# Autodesk Inventor assembly: POM_T5_11
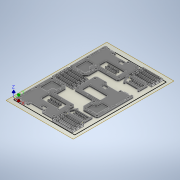
[picture p0: Inventor's stored thumbnail of the model, 180x180]
Saved by Autodesk Inventor 2022.3 (Build 263350000, 350)
## iProperties
Created: 2022-09-28
Part Number: POM_T5_11
Document SubType Name: Assembly
Designer: Masato
Author: Masato
## Documents named in this file (7)
- C:\Users\Masato\Documents\Inventor\Inventor for CIT Brains\SUSTAINA-OP\Cam\POM_T5\POM_T5_11.iam
- C:\Users\Masato\Documents\Inventor\Inventor for CIT Brains\SUSTAINA-OP\Cam\DisposableBoard.ipt
- C:\Users\Masato\Documents\Inventor\Inventor for CIT Brains\SUSTAINA-OP\UpperBody\Cockpit\Cockpit_carrier_board_frame.ipt
- C:\Users\Masato\Documents\Inventor\Inventor for CIT Brains\SUSTAINA-OP\UpperBody\Cockpit\Cockpit_side_frame.ipt
- C:\Users\Masato\Documents\Inventor\Inventor for CIT Brains\SUSTAINA-OP\UpperBody\Cockpit\Cockpit_side_frame_MIR.ipt
- C:\Users\Masato\Documents\Inventor\Inventor for CIT Brains\SUSTAINA-OP\OptionParts\DrillingJigs\Cockpit_carrier_board_frame_Jig.ipt
- C:\Users\Masato\Documents\Inventor\Inventor for CIT Brains\SUSTAINA-OP\OptionParts\DrillingJigs\Cockpit_side_frame_Jig.ipt
## Components (20 placed, 6 different names)
1. DisposableBoard:1 — フラッシュ:1, フラッシュ:2, フラッシュ:3, フラッシュ:4, フラッシュ:5, フラッシュ:6
2. Cockpit_side_frame:1 — メイト:7, フラッシュ:5, フラッシュ:6, フラッシュ:9, Flush:12, Mate:18, Mate:27, Mate:29, Flush:14, Mate:35
3. Cockpit_side_frame_MIR:1 — メイト:11, フラッシュ:9, Mate:19, Mate:28, Mate:30, Flush:16
4. Cockpit_side_frame:2 — Mate:15
5. Cockpit_side_frame_Jig:4 — Mate:26, Mate:28, Mate:30
6. Cockpit_side_frame_Jig:5 — Mate:25, Mate:27, Mate:29
7. Cockpit_carrier_board_frame:10 — Mate:36, Flush:15, Mate:43, Mate:44, Mate:45
8. Cockpit_carrier_board_frame:11 — Mate:38, Flush:17, Mate:46, Mate:47
9. Cockpit_side_frame_Jig:6 — Mate:41, Mate:44, Mate:45, Flush:19
10. Cockpit_side_frame_Jig:7 — Mate:42, Flush:19, Mate:47
11. Cockpit_carrier_board_frame_Jig:1 — Mate:13, Flush:12, Mate:18
12. Cockpit_carrier_board_frame_Jig:2
13. Cockpit_carrier_board_frame_Jig:3
14. Cockpit_carrier_board_frame_Jig:4 — Mate:19
15. Cockpit_carrier_board_frame_Jig:5 — Mate:34, Flush:14, Mate:35, Flush:18
16. Cockpit_carrier_board_frame_Jig:6
17. Cockpit_carrier_board_frame_Jig:7 — Flush:15, Mate:43
18. Cockpit_carrier_board_frame_Jig:8 — Mate:39, Flush:16, Flush:17, Flush:18
19. Cockpit_carrier_board_frame_Jig:9
20. Cockpit_carrier_board_frame_Jig:10 — Mate:46
## Component patterns: (4 elements, first: Cockpit_carrier_board_frame_Jig:1), (3 elements, first: Cockpit_carrier_board_frame_Jig:5), (3 elements, first: Cockpit_carrier_board_frame_Jig:8)
## Relationships (38: Mate 24, Flush 14)
- フラッシュ:1 [Flush]: DisposableBoard:1
- フラッシュ:2 [Flush]: DisposableBoard:1
- フラッシュ:3 [Flush]: DisposableBoard:1
- フラッシュ:4 [Flush]: DisposableBoard:1
- メイト:7 [Mate]: Cockpit_side_frame:1
- メイト:11 [Mate]: Cockpit_side_frame_MIR:1
- フラッシュ:5 [Flush] (-1.65 mm): DisposableBoard:1 ↔ Cockpit_side_frame:1
- フラッシュ:6 [Flush] (2 mm): DisposableBoard:1 ↔ Cockpit_side_frame:1
- フラッシュ:9 [Flush]: Cockpit_side_frame:1 ↔ Cockpit_side_frame_MIR:1
- Mate:13: Cockpit_carrier_board_frame_Jig:1
- Mate:15: Cockpit_side_frame:2
- Flush:12: Cockpit_side_frame:1 ↔ Cockpit_carrier_board_frame_Jig:1
- Mate:18 (2.1 mm): Cockpit_side_frame:1 ↔ Cockpit_carrier_board_frame_Jig:1
- Mate:19 (2.1 mm): Cockpit_side_frame_MIR:1 ↔ Cockpit_carrier_board_frame_Jig:4
- Mate:25: Cockpit_side_frame_Jig:5
- Mate:26: Cockpit_side_frame_Jig:4
- Mate:27 (7.225 mm): Cockpit_side_frame:1 ↔ Cockpit_side_frame_Jig:5
- Mate:28 (7.225 mm): Cockpit_side_frame_MIR:1 ↔ Cockpit_side_frame_Jig:4
- Mate:29 (13.425 mm): Cockpit_side_frame:1 ↔ Cockpit_side_frame_Jig:5
- Mate:30 (13.425 mm): Cockpit_side_frame_MIR:1 ↔ Cockpit_side_frame_Jig:4
- Mate:34: Cockpit_carrier_board_frame_Jig:5
- Flush:14: Cockpit_side_frame:1 ↔ Cockpit_carrier_board_frame_Jig:5
- Mate:35 (2.1 mm): Cockpit_side_frame:1 ↔ Cockpit_carrier_board_frame_Jig:5
- Mate:36: Cockpit_carrier_board_frame:10
- Flush:15: Cockpit_carrier_board_frame:10 ↔ Cockpit_carrier_board_frame_Jig:7
- Mate:38: Cockpit_carrier_board_frame:11
- Mate:39: Cockpit_carrier_board_frame_Jig:8
- Flush:16: Cockpit_side_frame_MIR:1 ↔ Cockpit_carrier_board_frame_Jig:8
- Flush:17: Cockpit_carrier_board_frame:11 ↔ Cockpit_carrier_board_frame_Jig:8
- Flush:18: Cockpit_carrier_board_frame_Jig:5 ↔ Cockpit_carrier_board_frame_Jig:8
- Mate:41: Cockpit_side_frame_Jig:6
- Mate:42: Cockpit_side_frame_Jig:7
- Mate:43 (2.1 mm): Cockpit_carrier_board_frame:10 ↔ Cockpit_carrier_board_frame_Jig:7
- Mate:44 (6.2071 mm): Cockpit_carrier_board_frame:10 ↔ Cockpit_side_frame_Jig:6
- Mate:45 (2.975 mm): Cockpit_carrier_board_frame:10 ↔ Cockpit_side_frame_Jig:6
- Mate:46 (2.1 mm): Cockpit_carrier_board_frame:11 ↔ Cockpit_carrier_board_frame_Jig:10
- Flush:19: Cockpit_side_frame_Jig:6 ↔ Cockpit_side_frame_Jig:7
- Mate:47 (2.1 mm): Cockpit_carrier_board_frame:11 ↔ Cockpit_side_frame_Jig:7
